# Autodesk Inventor assembly: Ensemble1
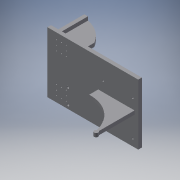
[picture p0: Inventor's stored thumbnail of the model, 180x180]
Saved by Autodesk Inventor 2017 (Build 210142000, 142)
## iProperties
Part Number: Ensemble1
Material: Générique
Document SubType Name: Assembly
Designer: Thomas
Author: Thomas
## Documents named in this file (5)
- C:\Users\Thomas\Documents\Modele 3D\FIRSTBOT\Ensemble1.iam
- C:\Users\Thomas\Documents\Modele 3D\FIRSTBOT\attache.ipt
- C:\Users\Thomas\Documents\Modele 3D\FIRSTBOT\base.ipt
- C:\Users\Thomas\Documents\Modele 3D\FIRSTBOT\latéral.ipt
- C:\Users\Thomas\Documents\Modele 3D\FIRSTBOT\roue_libre.ipt
## Components (5 placed, 4 different names)
1. attache:1 — Placage:1, Placage:2, Placage:3, Placage:4, Affleurement:3, Placage:5, Placage:6, Placage:7
2. base:1 — Placage:1, Placage:2, Placage:3, Affleurement:2, Affleurement:4, Placage:8, Placage:9
3. latéral:1 — Placage:4, Affleurement:2, Affleurement:3
4. latéral:2 — Placage:5, Placage:6, Placage:7
5. roue_libre:1 — Affleurement:4, Placage:8, Placage:9
## Relationships (12: Mate 9, Flush 3)
- Placage:1 [Mate]: attache:1 ↔ base:1
- Placage:2 [Mate]: attache:1 ↔ base:1
- Placage:3 [Mate]: attache:1 ↔ base:1
- Placage:4 [Mate]: attache:1 ↔ latéral:1
- Affleurement:2 [Flush]: base:1 ↔ latéral:1
- Affleurement:3 [Flush]: attache:1 ↔ latéral:1
- Placage:5 [Mate]: attache:1 ↔ latéral:2
- Placage:6 [Mate]: attache:1 ↔ latéral:2
- Placage:7 [Mate]: attache:1 ↔ latéral:2
- Affleurement:4 [Flush]: base:1 ↔ roue_libre:1
- Placage:8 [Mate]: base:1 ↔ roue_libre:1
- Placage:9 [Mate]: base:1 ↔ roue_libre:1
